# Autodesk Inventor assembly: 4xStack
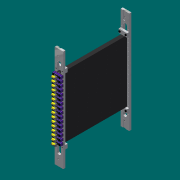
[picture p0: Inventor's stored thumbnail of the model, 180x180]
Saved by Autodesk Inventor 2016 SP1 (Build 200210100, 210)
## iProperties
Created: 2016-02-15
Part Number: 4xStack
Document SubType Name: Assembly
Designer: sawai
Author: sawai
## Documents named in this file (7)
- C:\Users\sawaiz\OneDrive\projects\scintillatorPanel\4xStack.iam
- C:\Users\sawaiz\OneDrive\projects\scintillatorPanel\scintillatorPanel.iam
- C:\Users\sawaiz\OneDrive\projects\scintillatorPanel\coluredSpacer.ipt
- C:\Users\sawaiz\OneDrive\projects\scintillatorPanel\mppcMount.ipt
- C:\Users\sawaiz\OneDrive\projects\scintillatorPanel\suppourtBlock.ipt
- C:\Users\sawaiz\OneDrive\projects\scintillatorPanel\4-40x0.5in.ipt
- C:\Users\sawaiz\OneDrive\projects\scintillatorPanel\scintillator.xlsx
## Components (38 placed, 5 different names)
1. mppcMount:1 — Mate:3, Mate:4, Mate:5, Mate:7, Flush:21, Flush:22, Symmetry:1, Symmetry:2, Symmetry:3, Mate:9, Flush:25, Mate:10, Flush:28
2. mppcMount:2 — Flush:21, Flush:22, Symmetry:1, Symmetry:2, Symmetry:3, Mate:8, Flush:24, Mate:11, Flush:27, Flush:30, Mate:26
3. suppourtBlock:1 — Mate:11, Flush:27, Flush:29, Mate:18, Mate:19, Mate:25
4. suppourtBlock:2 — Mate:10, Flush:28, Flush:29, Symmetry:4, Mate:12, Mate:13, Mate:20, Mate:21, Mate:22
5. suppourtBlock:3 — Mate:8, Flush:24, Flush:26, Symmetry:4, Mate:16, Mate:17, Mate:24, Mate:26
6. suppourtBlock:4 — Mate:9, Flush:25, Flush:26, Mate:14, Mate:15, Mate:23
7. 4-40x0.5in:1 — Flush:32, Mate:19, Mate:25
8. 4-40x0.5in:2 — Flush:32, Mate:18
9. 4-40x0.5in:3 — Mate:12, Flush:34, Mate:21
10. 4-40x0.5in:4 — Mate:13, Flush:34, Mate:20, Mate:22
11. 4-40x0.5in:5 — Mate:16, Flush:31
12. 4-40x0.5in:6 — Mate:17, Flush:31, Mate:24
13. 4-40x0.5in:7 — Mate:15, Flush:33
14. 4-40x0.5in:8 — Mate:14, Flush:33, Mate:23
15. scintillatorPanel:1 [sub-assembly] — Mate:3, Mate:4, Mate:5, Mate:6, Flush:20, Flush:30
16. scintillatorPanel:3 [sub-assembly]
17. scintillatorPanel:4 [sub-assembly]
18. scintillatorPanel:5 [sub-assembly]
19. scintillatorPanel:6 [sub-assembly]
20. scintillatorPanel:7 [sub-assembly]
21. scintillatorPanel:8 [sub-assembly]
22. scintillatorPanel:9 [sub-assembly]
23. scintillatorPanel:10 [sub-assembly]
24. scintillatorPanel:11 [sub-assembly]
25. scintillatorPanel:12 [sub-assembly]
26. scintillatorPanel:13 [sub-assembly]
27. scintillatorPanel:14 [sub-assembly]
28. scintillatorPanel:15 [sub-assembly]
29. scintillatorPanel:16 [sub-assembly]
30. scintillatorPanel:17 [sub-assembly]
31. coluredSpacer:1 — Mate:6, Flush:20, Mate:7
32. coluredSpacer:2
33. coluredSpacer:3
34. coluredSpacer:4
35. coluredSpacer:5
36. coluredSpacer:6
37. coluredSpacer:7
38. coluredSpacer:8
## Component patterns: (16 elements, first: scintillatorPanel:1), (8 elements, first: coluredSpacer:1)
## Relationships (42: Mate 24, Flush 14, Symmetry 4)
- Mate:3: mppcMount:1 ↔ scintillatorPanel:1
- Mate:4: mppcMount:1 ↔ scintillatorPanel:1
- Mate:5: mppcMount:1 ↔ scintillatorPanel:1
- Mate:6: scintillatorPanel:1 ↔ coluredSpacer:1
- Flush:20: scintillatorPanel:1 ↔ coluredSpacer:1
- Mate:7: mppcMount:1 ↔ coluredSpacer:1
- Flush:21: mppcMount:1 ↔ mppcMount:2
- Flush:22: mppcMount:1 ↔ mppcMount:2
- Symmetry:1: mppcMount:1 ↔ mppcMount:2
- Symmetry:2: mppcMount:1 ↔ mppcMount:2
- Symmetry:3: mppcMount:1 ↔ mppcMount:2
- Mate:8: mppcMount:2 ↔ suppourtBlock:3
- Flush:24: mppcMount:2 ↔ suppourtBlock:3
- Mate:9: mppcMount:1 ↔ suppourtBlock:4
- Flush:25: mppcMount:1 ↔ suppourtBlock:4
- Flush:26: suppourtBlock:3 ↔ suppourtBlock:4
- Mate:10: mppcMount:1 ↔ suppourtBlock:2
- Mate:11: mppcMount:2 ↔ suppourtBlock:1
- Flush:27: mppcMount:2 ↔ suppourtBlock:1
- Flush:28: mppcMount:1 ↔ suppourtBlock:2
- Flush:29: suppourtBlock:1 ↔ suppourtBlock:2
- Flush:30: mppcMount:2 ↔ scintillatorPanel:1
- Symmetry:4: suppourtBlock:2 ↔ suppourtBlock:3
- Mate:12: suppourtBlock:2 ↔ 4-40x0.5in:3
- Mate:13: suppourtBlock:2 ↔ 4-40x0.5in:4
- Mate:14: suppourtBlock:4 ↔ 4-40x0.5in:8
- Mate:15: suppourtBlock:4 ↔ 4-40x0.5in:7
- Mate:16: suppourtBlock:3 ↔ 4-40x0.5in:5
- Mate:17: suppourtBlock:3 ↔ 4-40x0.5in:6
- Flush:31: 4-40x0.5in:5 ↔ 4-40x0.5in:6
- Flush:32: 4-40x0.5in:1 ↔ 4-40x0.5in:2
- Flush:33: 4-40x0.5in:7 ↔ 4-40x0.5in:8
- Flush:34: 4-40x0.5in:3 ↔ 4-40x0.5in:4
- Mate:18: suppourtBlock:1 ↔ 4-40x0.5in:2
- Mate:19: suppourtBlock:1 ↔ 4-40x0.5in:1
- Mate:20: suppourtBlock:2 ↔ 4-40x0.5in:4
- Mate:21: suppourtBlock:2 ↔ 4-40x0.5in:3
- Mate:22: suppourtBlock:2 ↔ 4-40x0.5in:4
- Mate:23: suppourtBlock:4 ↔ 4-40x0.5in:8
- Mate:24: suppourtBlock:3 ↔ 4-40x0.5in:6
- Mate:25: suppourtBlock:1 ↔ 4-40x0.5in:1
- Mate:26 (-58.672 mm): mppcMount:2 ↔ suppourtBlock:3
## Named parameters: ScintillatorThickness = 10 mm, OpticalFiberClearence = 0.071 mm, ScintillatorEdgeClearence = 3 mm, ScintillatorWidth = 10 mm, ScintillatorHeight = 200 mm, ShallowTrackDepth = 1.142 mm, DeepTrackDepth = 5.571 mm, FiberEdgeOffsett = 5 mm, LoopLargeTrackRatio = 1.1, LoopSmallTrackDiameter = 90 mm, FiberSensorClerence = 0.5 mm, MountingScrewOffsett = 9 mm, LoopLength = 140 mm, silveringThickness = 0.2 mm, rubberizedCoating = 0.0508, mppcMountDepth = 6.35 mm, fingerCount = 16, stripeCount = 2
note: some values were not read from the file. Shown as the stored number, unit unknown: "rubberizedCoating".
